# Autodesk Inventor assembly: WheelMotor
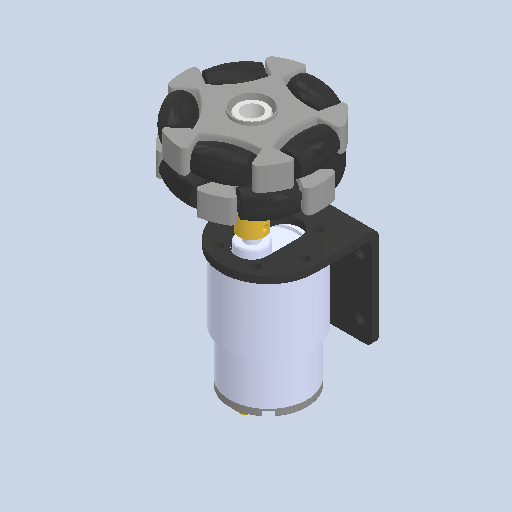
[picture p0: Inventor's stored thumbnail of the model, 512x512]
Saved by Autodesk Inventor 2025.1 (Build 291241000, 241)
## iProperties
Created: 2025-05-09
Part Number: WheelMotor
Document SubType Name: Assembly
Designer: User
Author: User
## Documents named in this file (6)
- D:\One Drive\OneDrive - Politeknik Sultan Salahuddin Abdul Aziz Shah\Documents\Inventor\RobosotPSA\WheelMotor.iam
- D:\One Drive\OneDrive - Politeknik Sultan Salahuddin Abdul Aziz Shah\Documents\Inventor\RobosotPSA\JGB37-520\JGB37-520\JGB37-520.ipt
- D:\One Drive\OneDrive - Politeknik Sultan Salahuddin Abdul Aziz Shah\Documents\Inventor\RobosotPSA\MM-JGB37 v4\MM-JGB37 v4\MM-JGB37 v4.ipt
- D:\One Drive\OneDrive - Politeknik Sultan Salahuddin Abdul Aziz Shah\Documents\Inventor\RobosotPSA\omni_ext.ipt
- D:\One Drive\OneDrive - Politeknik Sultan Salahuddin Abdul Aziz Shah\Documents\Inventor\RobosotPSA\geared motor brass coupling nut M12 nut 6mm shaft\geared motor brass coupling nut M12 nut 6mm shaft\geared moto.ipt
- D:\One Drive\OneDrive - Politeknik Sultan Salahuddin Abdul Aziz Shah\Documents\Inventor\RobosotPSA\58mm Omni-Directional Wheel\58mm Omni-Directional Wheel\58mm Omni-Directional Wheel.ipt
## Components (5 placed, 5 different names)
1. JGB37-520:1 — Mate:1, Mate:2, Mate:3, Mate:4, Mate:5
2. MM-JGB37 v4:1 — Mate:1, Mate:2, Mate:3
3. omni_ext:1 — Mate:6, Mate:8
4. geared moto:1 — Mate:4, Mate:5, Mate:6
5. 58mm Omni-Directional Wheel:1 — Mate:8
## Relationships (7: Mate 7)
- Mate:1: JGB37-520:1 ↔ MM-JGB37 v4:1
- Mate:2: JGB37-520:1 ↔ MM-JGB37 v4:1
- Mate:3: JGB37-520:1 ↔ MM-JGB37 v4:1
- Mate:4: JGB37-520:1 ↔ geared moto:1
- Mate:5: JGB37-520:1 ↔ geared moto:1
- Mate:6: omni_ext:1 ↔ geared moto:1
- Mate:8: omni_ext:1 ↔ 58mm Omni-Directional Wheel:1
